# Autodesk Inventor assembly: Serwo_z_widelcem
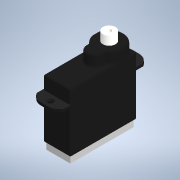
[picture p0: Inventor's stored thumbnail of the model, 180x180]
Saved by Autodesk Inventor 2022 (Build 260153000, 153)
## iProperties
Created: 2023-01-03
Part Number: Serwo_z_widelcem
Document SubType Name: Assembly
Designer: Kamil
Author: Kamil
## Documents named in this file (3)
- C:\MiniSumo koks\Serwo_z_widelcem.iam
- C:\MiniSumo koks\servo_mini_1370hd_cos.ipt
- C:\MiniSumo koks\Part6.ipt
## Components (2 placed, 2 different names)
1. servo_mini_1370hd_cos:1 — Flush:1
2. Part6:1 — Flush:1
## Relationships (3: Flush 3)
- Flush:1: servo_mini_1370hd_cos:1 ↔ Part6:1
- Flush:4 (7.5 mm)
- Flush:5 (-7.5 mm)
